# Autodesk Inventor assembly: MF85ZZ
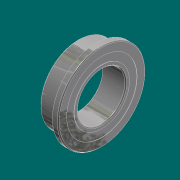
[picture p0: Inventor's stored thumbnail of the model, 180x180]
Saved by Autodesk Inventor 2016 (Build 200138000, 138)
## iProperties
Category: PARTsolutions
Company: NSK_RB
Created: 2016-04-26
Part Number: MF85ZZ
Catalog Web Link: www.cadenas.de
Description: Shielded Type ZZ-ZZS-
Vendor: NSK_RB
Document SubType Name: Assembly
Designer: psAdmin
Manufacturer: NSK_RB
Mass: 0.479397 g
Surface Area: 3.94786 cm^2
Volume: 0.0618577 cm^3
Density: 7.75 g/cm^3
PSOL_IDENT_0: {$CADENAS_DATA\23d-libs\nsk_rb\roller_bearings\deep_groove_bb\exstra_small_miniatur_bb\metric_design
PSOL_IDENT_1: _with_flange\shielded_type_zz_zzs_1_asmtab.prj},174 {VTYP=3D},{STYP=ASSTAB},{NB=MF85ZZ},{LINA=MF85ZZ
PSOL_IDENT_2: },{NN=Shielded Type ZZ-ZZS},{DATE=18.06.2013 02:54:37},{GEOMDATE=04.01.2008},{VERSION=},{LINEID=210}
PSOL_IDENT_3: ,{LINESUBID=-1},{WBVAR=}  {NB=MF85ZZ},{LINA=MF85ZZ},{KT=DUMMY},{IDNR=},{STAN=-},{ORDER=MF85ZZ},{SD=5
PSOL_IDENT_4: .0},{X=5.0},{D=8},{DD=8},{DD1=0.0},{D2=9.2},{DD2=9.2},{B=0.0},{B1=2.5},{CC1=0.0},{C2=0.6},{CC2=0.6},
PSOL_IDENT_5: {R=0.00},{R1=0.10},{DI1=5.80},{DI2=5.80},{SDE1=7.00},{SDE2=7.40},{CR1=310},{COR1=120},{CR2=31},{COR2=
PSOL_IDENT_6: 12.0},{LG=53000},{LO=63000},{DA=0.0},{DB=5.8},{RA=0.00},{RB=0.10},{MASS=0.41},{SC=1},{PPATH=shielded
PSOL_IDENT_7: _type_zz_zzs_asmtpl.prj}
NN: Shielded Type ZZ-ZZS
NB: MF85ZZ
NBSYN: $ORDER.
LINA: MF85ZZ
STAN: -
ORDER: MF85ZZ
SD: 5.0
D: 8
D2: 9.2
B1: 2.5
C2: 0.6
R1: 0.10
CR1: 310
COR1: 120
CR2: 31
COR2: 12.0
LG: 53000
DB: 5.8
RB: 0.10
MASS: 0.41
SUPPLIER: NSK_RB
ARTICLENO: MF85ZZ
BOMINFO: MF85ZZ
CREATOR: CADENAS GmbH
Title: MF85ZZ
Author: Cadenas PARTsolutions
## Documents named in this file (6)
- C:\Users\hiro\Documents\kenkyuu\二足\二足ver6.0\既製品\NSK_RB_MF85ZZ\MF85ZZ.iam
- C:\Users\hiro\Documents\kenkyuu\二足\二足ver6.0\既製品\NSK_RB_MF85ZZ\MF85ZZ Outer Ring.ipt
- C:\Users\hiro\Documents\kenkyuu\二足\二足ver6.0\既製品\NSK_RB_MF85ZZ\MF85ZZ Inner Ring.ipt
- C:\Users\hiro\Documents\kenkyuu\二足\二足ver6.0\既製品\NSK_RB_MF85ZZ\MF85ZZ Shield1.ipt
- C:\Users\hiro\Documents\kenkyuu\二足\二足ver6.0\既製品\NSK_RB_MF85ZZ\MF85ZZ Ball.ipt
- C:\Users\hiro\Documents\kenkyuu\二足\二足ver6.0\既製品\NSK_RB_MF85ZZ\MF85ZZ Shield2.ipt
## Components (21 placed, 5 different names)
1. MF85ZZ Outer Ring:1 — メイト:1, メイト:2
2. MF85ZZ Inner Ring:1
3. MF85ZZ Shield1:1 — メイト:1, メイト:2
4. MF85ZZ Ball:1
5. MF85ZZ Ball:2
6. MF85ZZ Ball:3
7. MF85ZZ Ball:4
8. MF85ZZ Ball:5
9. MF85ZZ Ball:6
10. MF85ZZ Ball:7
11. MF85ZZ Ball:8
12. MF85ZZ Ball:9
13. MF85ZZ Ball:10
14. MF85ZZ Ball:11
15. MF85ZZ Ball:12
16. MF85ZZ Ball:13
17. MF85ZZ Ball:14
18. MF85ZZ Ball:15
19. MF85ZZ Ball:16
20. MF85ZZ Ball:17
21. MF85ZZ Shield2:1
## Relationships (2: Mate 2)
- メイト:1 [Mate]: MF85ZZ Outer Ring:1 ↔ MF85ZZ Shield1:1
- メイト:2 [Mate]: MF85ZZ Outer Ring:1 ↔ MF85ZZ Shield1:1
